# Autodesk Inventor assembly: pulley_bracket_assem
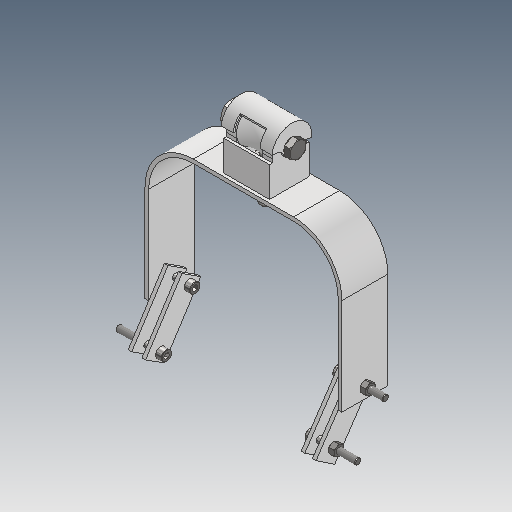
[picture p0: Inventor's stored thumbnail of the model, 512x512]
Saved by Autodesk Inventor 2025.2 (Build 292293000, 293)
## iProperties
Created: 2025-02-16
Part Number: pulley_bracket_assem
Document SubType Name: Assembly
Designer: email
Author: email
## Documents named in this file (13)
- C:\Users\email\Desktop\Projects\Capstone\4TB6\CAD_Model\thigh_mount_2\pulley_bracket_assem.iam
- C:\Users\email\Desktop\Projects\Capstone\4TB6\CAD_Model\thigh_mount_2\pulley_bracket.ipt
- C:\Users\email\Desktop\Projects\Capstone\4TB6\CAD_Model\thigh_mount_2\pulley_tab_right_A.ipt
- C:\Users\email\Desktop\Projects\Capstone\4TB6\CAD_Model\thigh_mount_2\pulley_tab_left_B.ipt
- C:\Users\email\Documents\Inventor\Content Center Files\R2025\en-US\CSN 02 1143  A\CSN 02 1143 - M5 x 0.8 x 35(1).ipt
- C:\Users\email\Documents\Inventor\Content Center Files\R2025\en-US\AS 1112 (2)\AS 1112 - M5  Type 5.ipt
- C:\Users\email\Desktop\Projects\Capstone\4TB6\CAD_Model\thigh_mount_2\pulley_base.ipt
- C:\Users\email\Desktop\Projects\Capstone\4TB6\CAD_Model\thigh_mount_2\pulley_bearing_cover.ipt
- C:\Users\email\Documents\Inventor\Content Center Files\R2025\en-US\BS 3469(2)\BS 3469 - 10 - 8 x 22 x 7.ipt
- C:\Users\email\Documents\Inventor\Content Center Files\R2025\en-US\AS 1110\AS 1110 - M8 x 50.ipt
- C:\Users\email\Documents\Inventor\Content Center Files\R2025\en-US\CSN 02 1143  A\CSN 02 1143 - M10 x 1.5 x 25(1).ipt
- C:\Users\email\Documents\Inventor\Content Center Files\R2025\en-US\AS 1112 (2)\AS 1112 - M10  Type 5.ipt
- C:\Users\email\Desktop\Projects\Capstone\4TB6\CAD_Model\thigh_mount_2\pulley_bearing_base_cover.ipt
## Components (23 placed, 12 different names)
1. pulley_bracket:1 — Mate:1, Mate:3, Mate:10, Mate:11, Mate:12, Mate:20, Mate:25, Mate:27, Mate:35, Mate:36, Mate:40, Angle:1
2. pulley_tab_right_A:1 — Mate:4, Mate:5, Mate:6, Mate:7, Mate:9
3. pulley_tab_right_A:2 — Mate:2, Mate:3, Mate:5, Mate:8, Mate:10, Mate:26
4. pulley_tab_left_B:1 — Mate:13, Mate:15, Mate:16, Mate:17, Mate:19
5. pulley_tab_left_B:2 — Mate:11, Mate:14, Mate:16, Mate:18, Mate:20, Mate:28
6. CSN 02 1143 A M5 x 35:1 — Mate:1, Mate:2, Mate:4, Mate:6, Mate:21
7. CSN 02 1143 A M5 x 35:2 — Mate:7, Mate:8, Mate:9, Mate:22
8. CSN 02 1143 A M5 x 35:3 — Mate:12, Mate:13, Mate:14, Mate:15, Mate:23
9. CSN 02 1143 A M5 x 35:4 — Mate:17, Mate:18, Mate:19, Mate:24
10. AS 1112 (2) - Metric M5  Type 5:1 — Mate:23, Mate:27
11. AS 1112 (2) - Metric M5  Type 5:2 — Mate:24, Mate:28
12. AS 1112 (2) - Metric M5  Type 5:3 — Mate:21, Mate:25
13. AS 1112 (2) - Metric M5  Type 5:4 — Mate:22, Mate:26
14. pulley_base:1 — Mate:35, Mate:36, Mate:37, Mate:38, Mate:41, Mate:42, Mate:43, Mate:45, Mate:47, Angle:1
15. pulley_bearing_cover:1 — Mate:33, Flush:1, Mate:43
16. BS 3469 (Metric) 10 - 8 x 22 x 7:1 — Mate:29, Mate:31
17. BS 3469 (Metric) 10 - 8 x 22 x 7:2 — Mate:29, Mate:30, Mate:31, Mate:32
18. BS 3469 (Metric) 10 - 8 x 22 x 7:3 — Mate:30, Mate:32, Mate:33, Flush:1, Mate:34
19. AS 1110 - Metric M8 x 50:1 — Mate:34, Mate:41, Mate:42, Mate:44, Mate:46
20. CSN 02 1143 A M10 x 25:1 — Mate:37, Mate:38, Mate:39
21. AS 1112 (2) - Metric M10  Type 5:1 — Mate:39, Mate:40
22. AS 1112 (2) - Metric M10  Type 5:2 — Mate:44, Mate:45
23. pulley_bearing_base_cover:1 — Mate:46, Mate:47
## Relationships (49: Mate 47, Flush 1, Angle 1)
- Mate:1: pulley_bracket:1 ↔ CSN 02 1143 A M5 x 35:1
- Mate:2: pulley_tab_right_A:2 ↔ CSN 02 1143 A M5 x 35:1
- Mate:3: pulley_bracket:1 ↔ pulley_tab_right_A:2
- Mate:4: pulley_tab_right_A:1 ↔ CSN 02 1143 A M5 x 35:1
- Mate:5 (8.5 mm): pulley_tab_right_A:1 ↔ pulley_tab_right_A:2
- Mate:6: pulley_tab_right_A:1 ↔ CSN 02 1143 A M5 x 35:1
- Mate:7: pulley_tab_right_A:1 ↔ CSN 02 1143 A M5 x 35:2
- Mate:8: pulley_tab_right_A:2 ↔ CSN 02 1143 A M5 x 35:2
- Mate:9: pulley_tab_right_A:1 ↔ CSN 02 1143 A M5 x 35:2
- Mate:10: pulley_bracket:1 ↔ pulley_tab_right_A:2
- Mate:11: pulley_bracket:1 ↔ pulley_tab_left_B:2
- Mate:12: pulley_bracket:1 ↔ CSN 02 1143 A M5 x 35:3
- Mate:13: pulley_tab_left_B:1 ↔ CSN 02 1143 A M5 x 35:3
- Mate:14: pulley_tab_left_B:2 ↔ CSN 02 1143 A M5 x 35:3
- Mate:15: pulley_tab_left_B:1 ↔ CSN 02 1143 A M5 x 35:3
- Mate:16 (8.5 mm): pulley_tab_left_B:1 ↔ pulley_tab_left_B:2
- Mate:17: pulley_tab_left_B:1 ↔ CSN 02 1143 A M5 x 35:4
- Mate:18: pulley_tab_left_B:2 ↔ CSN 02 1143 A M5 x 35:4
- Mate:19: pulley_tab_left_B:1 ↔ CSN 02 1143 A M5 x 35:4
- Mate:20: pulley_bracket:1 ↔ pulley_tab_left_B:2
- Mate:21: CSN 02 1143 A M5 x 35:1 ↔ AS 1112 (2) - Metric M5  Type 5:3
- Mate:22: CSN 02 1143 A M5 x 35:2 ↔ AS 1112 (2) - Metric M5  Type 5:4
- Mate:23: CSN 02 1143 A M5 x 35:3 ↔ AS 1112 (2) - Metric M5  Type 5:1
- Mate:24: CSN 02 1143 A M5 x 35:4 ↔ AS 1112 (2) - Metric M5  Type 5:2
- Mate:25: pulley_bracket:1 ↔ AS 1112 (2) - Metric M5  Type 5:3
- Mate:26: pulley_tab_right_A:2 ↔ AS 1112 (2) - Metric M5  Type 5:4
- Mate:27: pulley_bracket:1 ↔ AS 1112 (2) - Metric M5  Type 5:1
- Mate:28: pulley_tab_left_B:2 ↔ AS 1112 (2) - Metric M5  Type 5:2
- Mate:29: BS 3469 (Metric) 10 - 8 x 22 x 7:1 ↔ BS 3469 (Metric) 10 - 8 x 22 x 7:2
- Mate:30: BS 3469 (Metric) 10 - 8 x 22 x 7:2 ↔ BS 3469 (Metric) 10 - 8 x 22 x 7:3
- Mate:31: BS 3469 (Metric) 10 - 8 x 22 x 7:1 ↔ BS 3469 (Metric) 10 - 8 x 22 x 7:2
- Mate:32: BS 3469 (Metric) 10 - 8 x 22 x 7:2 ↔ BS 3469 (Metric) 10 - 8 x 22 x 7:3
- Mate:33: pulley_bearing_cover:1 ↔ BS 3469 (Metric) 10 - 8 x 22 x 7:3
- Flush:1: pulley_bearing_cover:1 ↔ BS 3469 (Metric) 10 - 8 x 22 x 7:3
- Mate:34: BS 3469 (Metric) 10 - 8 x 22 x 7:3 ↔ AS 1110 - Metric M8 x 50:1
- Mate:35: pulley_bracket:1 ↔ pulley_base:1
- Mate:36: pulley_bracket:1 ↔ pulley_base:1
- Mate:37: pulley_base:1 ↔ CSN 02 1143 A M10 x 25:1
- Mate:38: pulley_base:1 ↔ CSN 02 1143 A M10 x 25:1
- Mate:39: CSN 02 1143 A M10 x 25:1 ↔ AS 1112 (2) - Metric M10  Type 5:1
- Mate:40: pulley_bracket:1 ↔ AS 1112 (2) - Metric M10  Type 5:1
- Mate:41: pulley_base:1 ↔ AS 1110 - Metric M8 x 50:1
- Mate:42 (2 mm): pulley_base:1 ↔ AS 1110 - Metric M8 x 50:1
- Mate:43 (0.5 mm): pulley_base:1 ↔ pulley_bearing_cover:1
- Mate:44: AS 1110 - Metric M8 x 50:1 ↔ AS 1112 (2) - Metric M10  Type 5:2
- Mate:45 (2 mm): pulley_base:1 ↔ AS 1112 (2) - Metric M10  Type 5:2
- Mate:46: AS 1110 - Metric M8 x 50:1 ↔ pulley_bearing_base_cover:1
- Mate:47 (0.05 mm): pulley_base:1 ↔ pulley_bearing_base_cover:1
- Angle:1 (0 deg): pulley_bracket:1 ↔ pulley_base:1
